# Autodesk Inventor assembly: west coast drive base
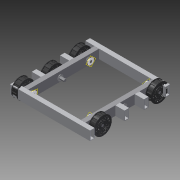
[picture p0: Inventor's stored thumbnail of the model, 180x180]
Saved by Autodesk Inventor 2015 (Build 190159000, 159)
## iProperties
Created: 2014-07-12
Part Number: west coast drive base
Document SubType Name: Assembly
Designer: admin
Author: admin
## Documents named in this file (6)
- C:\Users\Austin\Documents\GitHub\2014-2015\CAD\west coast drive\west coast drive base.iam
- C:\Users\Austin\Documents\GitHub\2014-2015\CAD\west coast drive\Wheel Vexpro 4in .iam
- C:\Users\Austin\Documents\GitHub\2014-2015\CAD\west coast drive\frame side assembly.iam
- C:\Users\Austin\Documents\GitHub\2014-2015\CAD\COTSParts\Structural\Aluminum Box Tube.ipt
- C:\Users\Austin\Documents\GitHub\2014-2015\CAD\west coast drive\Aluminum Box Tube.ipt
- C:\Users\Austin\Documents\GitHub\2014-2015\CAD\west coast drive\.5 inch hex axle center - Copy.ipt
## Components (10 placed, 4 different names)
1. frame side assembly:1 [sub-assembly] — Mate:2, Flush:1, Flush:3, Mate:4, Flush:5, Mate:7, Mate:8, Flush:7, Flush:8, Mate:9, Mate:10, Mate:11, Flush:11
2. frame side assembly:2 [sub-assembly] — Mate:3, Flush:2, Flush:4, Flush:6, Mate:5, Mate:6, Flush:9, Flush:10
3. Aluminum Box Tube:1 — Mate:2, Flush:1, Mate:3, Flush:2, Flush:3, Flush:4
4. Aluminum Box Tube:2 — Mate:4, Flush:5, Flush:6
5. Aluminum Box Tube:3 — Mate:8, Flush:7
6. Aluminum Box Tube:4 — Mate:7, Flush:8
7. Aluminum Box Tube:5 — Mate:6, Flush:10
8. Aluminum Box Tube:6 — Mate:5, Flush:9
9. .5 inch hex axle center - Copy:1 — Mate:9, Mate:10, Mate:11, Flush:11, Mate:12, Mate:13, Flush:12
10. Wheel Vexpro 4in :2 [sub-assembly] — Mate:12, Mate:13, Flush:12
## Relationships (24: Mate 12, Flush 12)
- Mate:2: frame side assembly:1 ↔ Aluminum Box Tube:1
- Flush:1 (50.8 mm): frame side assembly:1 ↔ Aluminum Box Tube:1
- Mate:3: frame side assembly:2 ↔ Aluminum Box Tube:1
- Flush:2: frame side assembly:2 ↔ Aluminum Box Tube:1
- Flush:3: frame side assembly:1 ↔ Aluminum Box Tube:1
- Flush:4 (50.8 mm): frame side assembly:2 ↔ Aluminum Box Tube:1
- Mate:4: frame side assembly:1 ↔ Aluminum Box Tube:2
- Flush:5: frame side assembly:1 ↔ Aluminum Box Tube:2
- Flush:6 (50.8 mm): frame side assembly:2 ↔ Aluminum Box Tube:2
- Mate:5: frame side assembly:2 ↔ Aluminum Box Tube:6
- Mate:6: frame side assembly:2 ↔ Aluminum Box Tube:5
- Mate:7: frame side assembly:1 ↔ Aluminum Box Tube:4
- Mate:8: frame side assembly:1 ↔ Aluminum Box Tube:3
- Flush:7: frame side assembly:1 ↔ Aluminum Box Tube:3
- Flush:8: frame side assembly:1 ↔ Aluminum Box Tube:4
- Flush:9: frame side assembly:2 ↔ Aluminum Box Tube:6
- Flush:10: frame side assembly:2 ↔ Aluminum Box Tube:5
- Mate:9: frame side assembly:1 ↔ .5 inch hex axle center - Copy:1
- Mate:10: frame side assembly:1 ↔ .5 inch hex axle center - Copy:1
- Mate:11: frame side assembly:1 ↔ .5 inch hex axle center - Copy:1
- Flush:11 (-25.4 mm): frame side assembly:1 ↔ .5 inch hex axle center - Copy:1
- Mate:12: .5 inch hex axle center - Copy:1 ↔ Wheel Vexpro 4in :2
- Mate:13: .5 inch hex axle center - Copy:1 ↔ Wheel Vexpro 4in :2
- Flush:12: .5 inch hex axle center - Copy:1 ↔ Wheel Vexpro 4in :2
